# Autodesk Inventor assembly: Frame Horizontals
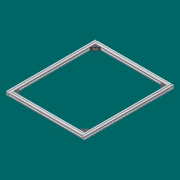
[picture p0: Inventor's stored thumbnail of the model, 180x180]
Saved by Autodesk Inventor 2016 SP1 (Build 200210100, 210)
## iProperties
Created: 2015-06-02
Part Number: Frame Horizontals
Document SubType Name: Assembly
Designer: Sawaiz Syed
Author: Sawaiz Syed
## Documents named in this file (4)
- C:\Users\Sawaiz\OneDrive\projects\modularRICH\testMount\frame\frameHorizontal.iam
- C:\Users\Sawaiz\OneDrive\projects\modularRICH\testMount\frame\hfs5-2020BeamAxisBeam.ipt
- C:\Users\Sawaiz\OneDrive\projects\modularRICH\testMount\frame\hfs5-2020OrthagonalBeamWidth.ipt
- C:\Users\Sawaiz\OneDrive\projects\modularRICH\testMount\frame\angleBracket.iam
## Components (8 placed, 3 different names)
1. hfs5-2020BeamAxisBeam:1 — Angle:2, Angle:3, Flush:3, Flush:4, Mate:3, Mate:4, Mate:9, Mate:11, Flush:8
2. hfs5-2020BeamAxisBeam:2 — Angle:1, Angle:4, Mate:1, Flush:1, Flush:2, Mate:2, Mate:10, Flush:7, Flush:10
3. hfs5-2020OrthagonalBeamWidth:3 — Flush:6, Mate:5, Mate:6, Mate:11, Flush:7
4. hfs5-2020OrthagonalBeamWidth:4 — Flush:5, Mate:7, Mate:8, Mate:9, Mate:10, Flush:8, Flush:9, Flush:10
5. angleBracket:1 [sub-assembly] — Angle:1, Mate:1, Flush:1, Mate:7, Flush:9
6. angleBracket:2 [sub-assembly] — Angle:2, Flush:4, Mate:4, Flush:5, Mate:8
7. angleBracket:3 [sub-assembly] — Angle:4, Flush:2, Mate:2, Mate:6
8. angleBracket:4 [sub-assembly] — Angle:3, Flush:3, Mate:3, Flush:6, Mate:5
## Relationships (25: Mate 11, Flush 10, Angle 4)
- Angle:1 (0 deg): hfs5-2020BeamAxisBeam:2 ↔ angleBracket:1
- Angle:2 (0 deg): hfs5-2020BeamAxisBeam:1 ↔ angleBracket:2
- Angle:3 (0 deg): hfs5-2020BeamAxisBeam:1 ↔ angleBracket:4
- Angle:4 (0 deg): hfs5-2020BeamAxisBeam:2 ↔ angleBracket:3
- Mate:1: hfs5-2020BeamAxisBeam:2 ↔ angleBracket:1
- Flush:1: hfs5-2020BeamAxisBeam:2 ↔ angleBracket:1
- Flush:2: hfs5-2020BeamAxisBeam:2 ↔ angleBracket:3
- Flush:3: hfs5-2020BeamAxisBeam:1 ↔ angleBracket:4
- Flush:4: hfs5-2020BeamAxisBeam:1 ↔ angleBracket:2
- Mate:2: hfs5-2020BeamAxisBeam:2 ↔ angleBracket:3
- Mate:3: hfs5-2020BeamAxisBeam:1 ↔ angleBracket:4
- Mate:4: hfs5-2020BeamAxisBeam:1 ↔ angleBracket:2
- Flush:5: hfs5-2020OrthagonalBeamWidth:4 ↔ angleBracket:2
- Flush:6: hfs5-2020OrthagonalBeamWidth:3 ↔ angleBracket:4
- Mate:5: hfs5-2020OrthagonalBeamWidth:3 ↔ angleBracket:4
- Mate:6: hfs5-2020OrthagonalBeamWidth:3 ↔ angleBracket:3
- Mate:7: hfs5-2020OrthagonalBeamWidth:4 ↔ angleBracket:1
- Mate:8: hfs5-2020OrthagonalBeamWidth:4 ↔ angleBracket:2
- Mate:9: hfs5-2020BeamAxisBeam:1 ↔ hfs5-2020OrthagonalBeamWidth:4
- Mate:10: hfs5-2020BeamAxisBeam:2 ↔ hfs5-2020OrthagonalBeamWidth:4
- Mate:11: hfs5-2020BeamAxisBeam:1 ↔ hfs5-2020OrthagonalBeamWidth:3
- Flush:7: hfs5-2020BeamAxisBeam:2 ↔ hfs5-2020OrthagonalBeamWidth:3
- Flush:8: hfs5-2020BeamAxisBeam:1 ↔ hfs5-2020OrthagonalBeamWidth:4
- Flush:9: hfs5-2020OrthagonalBeamWidth:4 ↔ angleBracket:1
- Flush:10: hfs5-2020BeamAxisBeam:2 ↔ hfs5-2020OrthagonalBeamWidth:4
